# Autodesk Inventor assembly: Neck_Base
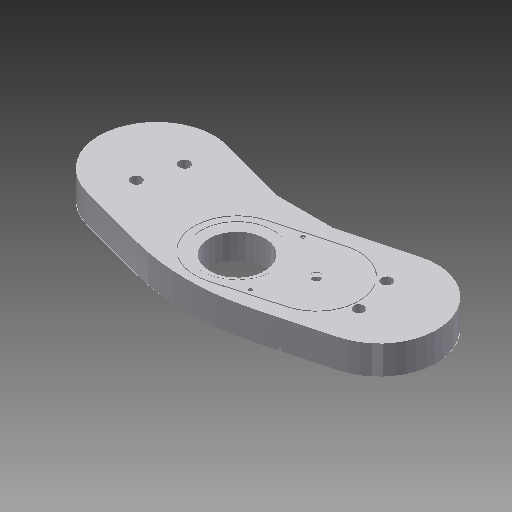
[picture p0: Inventor's stored thumbnail of the model, 512x512]
Saved by Autodesk Inventor 2017 SP1 (Build 210196100, 196)
## iProperties
Created: 2018-03-03
Part Number: Neck_Base
Document SubType Name: Assembly
Designer: Zach
Author: Zach
## Documents named in this file (2)
- C:\Users\Zach\Documents\GitHub\tr1_description\meshes\Visual Assembly\Neck_Base.iam
- C:\Users\Zach\Desktop\Neck_Base.ipt
## Components (1 placed, 1 different names)
1. Neck_Base:1 — Mate:1, Flush:1, Angle:1
## Relationships (3: Mate 1, Flush 1, Angle 1)
- Mate:1: Neck_Base:1
- Flush:1 (-20 mm): Neck_Base:1
- Angle:1 (180 deg): Neck_Base:1
